# Autodesk Inventor assembly: Left_Arm
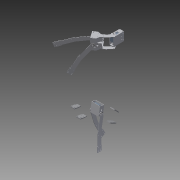
[picture p0: Inventor's stored thumbnail of the model, 180x180]
Saved by Autodesk Inventor 2013 (Build 170138000, 138)
## iProperties
Created: 2014-05-07
Part Number: Left_Arm
Document SubType Name: Assembly
Designer: andou
Mass: 429.088 g
Surface Area: 1516.71 cm^2
Volume: 223.56 cm^3
Density: 1.91934 g/cm^3
Author: andou
## Documents named in this file (16)
- C:\Users\andou\Documents\Inventor\RoboticsProject\project_4\Robot\Arm\Left_Arm\Left_Arm.iam
- C:\Users\andou\Documents\Inventor\RoboticsProject\project_4\Robot\All Common\Serial_Case.ipt
- C:\Users\andou\Documents\Inventor\RoboticsProject\project_4\Robot\Arm\KRS-2542HV.ipt
- C:\Users\andou\Documents\Inventor\RoboticsProject\project_4\Robot\Free_Horn\Free_Horn.iam
- C:\Users\andou\Documents\Inventor\RoboticsProject\project_4\Robot\All Common\Low_Height_Horn.ipt
- C:\Users\andou\Documents\Inventor\RoboticsProject\project_4\Robot\Arm\Horn_Spacer.ipt
- C:\Users\andou\Documents\Inventor\RoboticsProject\project_4\Robot\All Common\Washer(M4).ipt
- C:\Users\andou\Documents\Inventor\RoboticsProject\project_4\Robot\All Common\Nylon_Nat(M4).ipt
- C:\Users\andou\Documents\Inventor\RoboticsProject\project_4\Robot\All Common\Cap(M4-15).ipt
- C:\Users\andou\Documents\Inventor\RoboticsProject\project_4\Robot\All Common\Cap(M3-6).ipt
- C:\Users\andou\Documents\Inventor\RoboticsProject\project_4\Robot\Arm\Arm_Link.ipt
- C:\Users\andou\Documents\Inventor\RoboticsProject\project_4\Robot\Arm\Arm_Link_Shim.ipt
- C:\Users\andou\Documents\Inventor\RoboticsProject\project_4\Robot\Arm\Pitch_Serial_Case.ipt
- C:\Users\andou\Documents\Inventor\RoboticsProject\project_4\Robot\Arm\Arm_MiniLink.ipt
- C:\Users\andou\Documents\Inventor\RoboticsProject\project_4\Robot\Arm\Arm_MiniLink_Shim.ipt
- C:\Users\andou\Documents\Inventor\RoboticsProject\project_4\Robot\Arm\Yaw_Serial_Case.ipt
## Components (40 placed, 15 different names)
1. Free_Horn:1 [sub-assembly] — 挿入:15, 挿入:124, 挿入:137, 挿入:138
2. KRS-2542HV:1 — 挿入:8, 挿入:109, 挿入:110
3. Low_Height_Horn:1 — 挿入:8, 挿入:11, 挿入:12
4. Horn_Spacer:1 — 挿入:11, 挿入:12, 挿入:16, 挿入:139, 挿入:140
5. Washer(M4):1 — 挿入:14, 挿入:111
6. Nylon_Nat(M4):1 — 挿入:14
7. Cap(M4-15):1 — 挿入:15
8. Cap(M3-6):1 — 挿入:16
9. KRS-2542HV:2 — 挿入:25, 挿入:131, 挿入:132
10. Horn_Spacer:2 — 挿入:21, 挿入:23, 挿入:26, 挿入:44, 挿入:45
11. Free_Horn:2 [sub-assembly] — 挿入:46, 挿入:114, 挿入:142
12. Cap(M3-6):2 — 挿入:23
13. Cap(M4-15):2 — 挿入:114
14. Low_Height_Horn:2 — 挿入:21, 挿入:25, 挿入:26
15. Washer(M4):2 — 挿入:22, 挿入:141
16. Nylon_Nat(M4):2 — 挿入:22
17. Arm_Link:3 — 挿入:46, 挿入:48, 挿入:55
18. Arm_Link:4 — 挿入:44, 挿入:45, 挿入:105, 挿入:106
19. Serial_Case:3 — 挿入:33, 挿入:34, 挿入:37, 挿入:38, 挿入:103, 挿入:104, 挿入:112, 挿入:113
20. Nylon_Nat(M4):3 — 挿入:36
21. Washer(M4):3 — 挿入:36, 挿入:37
22. Low_Height_Horn:3 — 挿入:31, 挿入:32
23. Cap(M4-15):3 — 挿入:35
24. Cap(M3-6):3 — 挿入:39
25. Free_Horn:3 [sub-assembly] — 挿入:35, 挿入:38, 挿入:82, 挿入:85
26. Horn_Spacer:3 — 挿入:31, 挿入:39, 挿入:83, 挿入:84
27. KRS-2542HV:3 — 挿入:32, 挿入:33, 挿入:34
28. Arm_Link_Shim:4 — 挿入:48, 挿入:55, 挿入:112, 挿入:113
29. Arm_Link:5 — 挿入:82, 挿入:85, 挿入:107, 挿入:108
30. Arm_Link:6 — 挿入:83, 挿入:84, 挿入:99, 挿入:100, メイト:1
31. Arm_Link_Shim:6 — 挿入:99, 挿入:100
32. Arm_Link_Shim:7 — 挿入:103, 挿入:104, 挿入:105, 挿入:106
33. Arm_Link_Shim:8 — 挿入:107, 挿入:108, メイト:1
34. Pitch_Serial_Case:1 — 挿入:109, 挿入:110, 挿入:111, 挿入:124
35. Arm_MiniLink:1 — 挿入:126, 挿入:130, 挿入:137, 挿入:138
36. Arm_MiniLink:2 — 挿入:125, 挿入:128, 挿入:139, 挿入:140
37. Arm_MiniLink_Shim:1 — 挿入:125, 挿入:127, 挿入:128, 挿入:129
38. Arm_MiniLink_Shim:2 — 挿入:126, 挿入:130, 挿入:135, 挿入:136
39. Arm_MiniLink_Shim:3 — 挿入:127, 挿入:129, 挿入:133, 挿入:134
40. Yaw_Serial_Case:1 — 挿入:131, 挿入:132, 挿入:133, 挿入:134, 挿入:135, 挿入:136, 挿入:141, 挿入:142
## Relationships (63: Insert 62, Mate 1)
- 挿入:8 [Insert]: KRS-2542HV:1 ↔ Low_Height_Horn:1
- 挿入:11 [Insert]: Low_Height_Horn:1 ↔ Horn_Spacer:1
- 挿入:12 [Insert]: Low_Height_Horn:1 ↔ Horn_Spacer:1
- 挿入:14 [Insert]: Washer(M4):1 ↔ Nylon_Nat(M4):1
- 挿入:15 [Insert]: Free_Horn:1 ↔ Cap(M4-15):1
- 挿入:16 [Insert]: Horn_Spacer:1 ↔ Cap(M3-6):1
- 挿入:21 [Insert]: Horn_Spacer:2 ↔ Low_Height_Horn:2
- 挿入:22 [Insert]: Washer(M4):2 ↔ Nylon_Nat(M4):2
- 挿入:23 [Insert]: Horn_Spacer:2 ↔ Cap(M3-6):2
- 挿入:25 [Insert]: KRS-2542HV:2 ↔ Low_Height_Horn:2
- 挿入:26 [Insert]: Horn_Spacer:2 ↔ Low_Height_Horn:2
- 挿入:31 [Insert]: Low_Height_Horn:3 ↔ Horn_Spacer:3
- 挿入:32 [Insert]: Low_Height_Horn:3 ↔ KRS-2542HV:3
- 挿入:33 [Insert]: Serial_Case:3 ↔ KRS-2542HV:3
- 挿入:34 [Insert]: Serial_Case:3 ↔ KRS-2542HV:3
- 挿入:35 [Insert]: Cap(M4-15):3 ↔ Free_Horn:3
- 挿入:36 [Insert]: Nylon_Nat(M4):3 ↔ Washer(M4):3
- 挿入:37 [Insert]: Serial_Case:3 ↔ Washer(M4):3
- 挿入:38 [Insert]: Serial_Case:3 ↔ Free_Horn:3
- 挿入:39 [Insert]: Cap(M3-6):3 ↔ Horn_Spacer:3
- 挿入:44 [Insert]: Horn_Spacer:2 ↔ Arm_Link:4
- 挿入:45 [Insert]: Horn_Spacer:2 ↔ Arm_Link:4
- 挿入:46 [Insert]: Free_Horn:2 ↔ Arm_Link:3
- 挿入:48 [Insert]: Arm_Link:3 ↔ Arm_Link_Shim:4
- 挿入:55 [Insert]: Arm_Link:3 ↔ Arm_Link_Shim:4
- 挿入:82 [Insert]: Free_Horn:3 ↔ Arm_Link:5
- 挿入:83 [Insert]: Horn_Spacer:3 ↔ Arm_Link:6
- 挿入:84 [Insert]: Horn_Spacer:3 ↔ Arm_Link:6
- 挿入:85 [Insert]: Free_Horn:3 ↔ Arm_Link:5
- 挿入:99 [Insert]: Arm_Link:6 ↔ Arm_Link_Shim:6
- 挿入:100 [Insert]: Arm_Link:6 ↔ Arm_Link_Shim:6
- 挿入:103 [Insert]: Serial_Case:3 ↔ Arm_Link_Shim:7
- 挿入:104 [Insert]: Serial_Case:3 ↔ Arm_Link_Shim:7
- 挿入:105 [Insert]: Arm_Link:4 ↔ Arm_Link_Shim:7
- 挿入:106 [Insert]: Arm_Link:4 ↔ Arm_Link_Shim:7
- 挿入:107 [Insert]: Arm_Link:5 ↔ Arm_Link_Shim:8
- 挿入:108 [Insert]: Arm_Link:5 ↔ Arm_Link_Shim:8
- 挿入:109 [Insert]: KRS-2542HV:1 ↔ Pitch_Serial_Case:1
- 挿入:110 [Insert]: KRS-2542HV:1 ↔ Pitch_Serial_Case:1
- 挿入:111 [Insert]: Washer(M4):1 ↔ Pitch_Serial_Case:1
- 挿入:112 [Insert]: Serial_Case:3 ↔ Arm_Link_Shim:4
- 挿入:113 [Insert]: Serial_Case:3 ↔ Arm_Link_Shim:4
- 挿入:114 [Insert]: Free_Horn:2 ↔ Cap(M4-15):2
- 挿入:124 [Insert]: Free_Horn:1 ↔ Pitch_Serial_Case:1
- メイト:1 [Mate] (2.821 mm): Arm_Link:6 ↔ Arm_Link_Shim:8
- 挿入:125 [Insert]: Arm_MiniLink:2 ↔ Arm_MiniLink_Shim:1
- 挿入:126 [Insert]: Arm_MiniLink:1 ↔ Arm_MiniLink_Shim:2
- 挿入:127 [Insert]: Arm_MiniLink_Shim:1 ↔ Arm_MiniLink_Shim:3
- 挿入:128 [Insert]: Arm_MiniLink:2 ↔ Arm_MiniLink_Shim:1
- 挿入:129 [Insert]: Arm_MiniLink_Shim:1 ↔ Arm_MiniLink_Shim:3
- 挿入:130 [Insert]: Arm_MiniLink:1 ↔ Arm_MiniLink_Shim:2
- 挿入:131 [Insert]: KRS-2542HV:2 ↔ Yaw_Serial_Case:1
- 挿入:132 [Insert]: KRS-2542HV:2 ↔ Yaw_Serial_Case:1
- 挿入:133 [Insert]: Arm_MiniLink_Shim:3 ↔ Yaw_Serial_Case:1
- 挿入:134 [Insert]: Arm_MiniLink_Shim:3 ↔ Yaw_Serial_Case:1
- 挿入:135 [Insert]: Arm_MiniLink_Shim:2 ↔ Yaw_Serial_Case:1
- 挿入:136 [Insert]: Arm_MiniLink_Shim:2 ↔ Yaw_Serial_Case:1
- 挿入:137 [Insert]: Free_Horn:1 ↔ Arm_MiniLink:1
- 挿入:138 [Insert]: Free_Horn:1 ↔ Arm_MiniLink:1
- 挿入:139 [Insert]: Horn_Spacer:1 ↔ Arm_MiniLink:2
- 挿入:140 [Insert]: Horn_Spacer:1 ↔ Arm_MiniLink:2
- 挿入:141 [Insert]: Washer(M4):2 ↔ Yaw_Serial_Case:1
- 挿入:142 [Insert]: Free_Horn:2 ↔ Yaw_Serial_Case:1
